# Autodesk Inventor assembly: gear_box_base
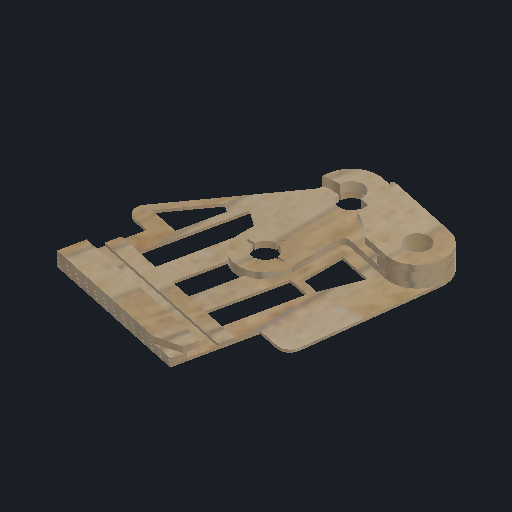
[picture p0: Inventor's stored thumbnail of the model, 512x512]
Saved by Autodesk Inventor 2026.3 (Build 303398000, 398)
## iProperties
Created: 2025-09-25
Part Number: gear_box_base
Document SubType Name: Assembly
Designer: hibik
Author: hibik
## Documents named in this file (7)
- D:\model\D2_Conveyor_2026\power_module\gear_box_base.iam
- D:\model\D2_Conveyor_2026\power_module\gear_plate_1.ipt
- D:\model\D2_Conveyor_2026\power_module\gear_plate_2.ipt
- D:\model\D2_Conveyor_2026\power_module\gear_plate_base.ipt
- D:\model\D2_Conveyor_2026\power_module\connector.ipt
- D:\model\D2_Conveyor_2026\power_module\gear_plate_3.ipt
- D:\model\D2_Conveyor_2026\power_module\stopper.ipt
## Components (8 placed, 6 different names)
1. gear_plate_1:1 — 挿入:5, 挿入:6, 挿入:7, 角度:1
2. gear_plate_base:1 — 挿入:5, 挿入:6, メイト:1, フラッシュ:1, フラッシュ:2, メイト:2, フラッシュ:3, フラッシュ:4
3. connector:1 — メイト:1, フラッシュ:1, フラッシュ:2
4. gear_plate_2:2 — 挿入:7, 挿入:8, 角度:1, 角度:2
5. gear_plate_3:1 — 挿入:8, 角度:2
6. connector:2 — メイト:2, フラッシュ:3, フラッシュ:4, メイト:3, フラッシュ:5, フラッシュ:6
7. connector:3 — メイト:3, フラッシュ:5, フラッシュ:6, メイト:4, フラッシュ:7, フラッシュ:8
8. stopper:1 — メイト:4, フラッシュ:7, フラッシュ:8
## Relationships (18: Flush 8, Insert 4, Mate 4, Angle 2)
- 挿入:5 [Insert]: gear_plate_1:1 ↔ gear_plate_base:1
- 挿入:6 [Insert]: gear_plate_1:1 ↔ gear_plate_base:1
- 挿入:7 [Insert]: gear_plate_1:1 ↔ gear_plate_2:2
- 挿入:8 [Insert]: gear_plate_2:2 ↔ gear_plate_3:1
- 角度:1 [Angle] (0 deg): gear_plate_1:1 ↔ gear_plate_2:2
- 角度:2 [Angle] (0 deg): gear_plate_2:2 ↔ gear_plate_3:1
- メイト:1 [Mate]: gear_plate_base:1 ↔ connector:1
- フラッシュ:1 [Flush]: gear_plate_base:1 ↔ connector:1
- フラッシュ:2 [Flush]: gear_plate_base:1 ↔ connector:1
- メイト:2 [Mate]: gear_plate_base:1 ↔ connector:2
- フラッシュ:3 [Flush]: gear_plate_base:1 ↔ connector:2
- フラッシュ:4 [Flush]: gear_plate_base:1 ↔ connector:2
- メイト:3 [Mate]: connector:2 ↔ connector:3
- フラッシュ:5 [Flush]: connector:2 ↔ connector:3
- フラッシュ:6 [Flush]: connector:2 ↔ connector:3
- メイト:4 [Mate]: connector:3 ↔ stopper:1
- フラッシュ:7 [Flush]: connector:3 ↔ stopper:1
- フラッシュ:8 [Flush]: connector:3 ↔ stopper:1
